# Autodesk Inventor assembly: Assembly1
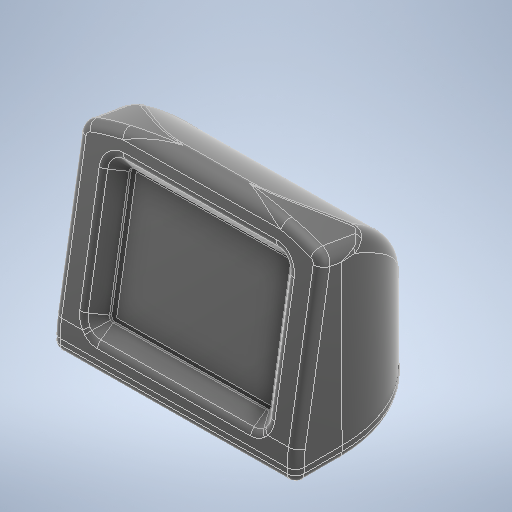
[picture p0: Inventor's stored thumbnail of the model, 512x512]
Saved by Autodesk Inventor 2025 (Build 290162000, 162)
## iProperties
Created: 2024-12-23
Part Number: Assembly1
Document SubType Name: Assembly
Designer: tvoko
Author: tvoko
## Documents named in this file (6)
- C:\Users\tvoko\Documents\Inventor\Misc-Projects\DesktopMazeBot\Hardware\Assembly1.iam
- C:\Users\tvoko\Documents\Inventor\Misc-Projects\DesktopMazeBot\Hardware\Buyouts\2090 2.8in TFT Cap Touch.ipt
- C:\Users\tvoko\Documents\School\Fall 2024\Senior Design Pt 1\Lab 1\Buyouts\5323 Feather ESP32-S3\5323 Feather ESP32-S3.ipt
- C:\Users\tvoko\Documents\Inventor\Misc-Projects\DesktopMazeBot\Hardware\Top.ipt
- C:\Users\tvoko\Documents\Inventor\Content Center Files\R2025\en-US\ISO 4762(2)\ISO 4762 - M3 x 5ISO.ipt
- C:\Users\tvoko\Documents\Inventor\Misc-Projects\DesktopMazeBot\Hardware\Bottom.ipt
## Components (6 placed, 5 different names)
1. 2090 2.8in TFT Cap Touch:1 — Mate:1, Mate:2, Mate:5, Mate:6, Mate:7
2. 5323 Feather ESP32-S3:1 — Mate:9, Mate:10
3. Top:1 — Mate:1, Mate:2, Mate:3, Mate:4, Mate:7, Mate:8
4. ISO 4762 M3 x 5:1 — Mate:3, Mate:5
5. ISO 4762 M3 x 5:2 — Mate:4, Mate:6
6. Bottom:1 — Mate:8, Mate:9, Mate:10
## Relationships (10: Mate 10)
- Mate:1: 2090 2.8in TFT Cap Touch:1 ↔ Top:1
- Mate:2: 2090 2.8in TFT Cap Touch:1 ↔ Top:1
- Mate:3: Top:1 ↔ ISO 4762 M3 x 5:1
- Mate:4: Top:1 ↔ ISO 4762 M3 x 5:2
- Mate:5: 2090 2.8in TFT Cap Touch:1 ↔ ISO 4762 M3 x 5:1
- Mate:6: 2090 2.8in TFT Cap Touch:1 ↔ ISO 4762 M3 x 5:2
- Mate:7: 2090 2.8in TFT Cap Touch:1 ↔ Top:1
- Mate:8: Top:1 ↔ Bottom:1
- Mate:9: 5323 Feather ESP32-S3:1 ↔ Bottom:1
- Mate:10: 5323 Feather ESP32-S3:1 ↔ Bottom:1
